# Autodesk Inventor assembly: S1702_EnsembleManetteTotal
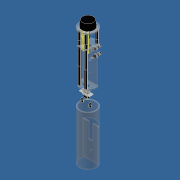
[picture p0: Inventor's stored thumbnail of the model, 180x180]
Saved by Autodesk Inventor 2015 SP2 (Build 190223200, 223)
## iProperties
Created: 2017-12-07
Part Number: S1702_EnsembleManetteTotal
Project: Nom Projet
Description: Ens. Nom Ensemble
Document SubType Name: Assembly
Designer: Benoit.CURCHOD2
Author: Benoit.CURCHOD2
## Documents named in this file (24)
- Z:\COMMUN\4. Projets\2. Projets PO\S1702_Circuit_sport\14_Conception 3D\Manette\Final\S1702_EnsembleManetteTotal.iam
- Z:\COMMUN\4. Projets\2. Projets PO\S1702_Circuit_sport\14_Conception 3D\Manette\Final\S1702_couverclebas.ipt
- Z:\COMMUN\4. Projets\2. Projets PO\S1702_Circuit_sport\14_Conception 3D\Manette\Final\Bouton poussoir NO.iam
- Z:\COMMUN\4. Projets\2. Projets PO\S1702_Circuit_sport\14_Conception 3D\Manette\Final\Bouton.ipt
- Z:\COMMUN\4. Projets\2. Projets PO\S1702_Circuit_sport\14_Conception 3D\Manette\Final\Capuchon.ipt
- Z:\COMMUN\4. Projets\2. Projets PO\S1702_Circuit_sport\14_Conception 3D\Manette\Final\Entretoise 12 x M3.ipt
- Z:\COMMUN\4. Projets\2. Projets PO\S1702_Circuit_sport\14_Conception 3D\Manette\Final\Entretoise 25.ipt
- Z:\COMMUN\4. Projets\2. Projets PO\S1702_Circuit_sport\14_Conception 3D\Manette\Final\Entretoise 50.ipt
- Z:\COMMUN\4. Projets\2. Projets PO\S1702_Circuit_sport\14_Conception 3D\Manette\Final\Molette.ipt
- Z:\COMMUN\4. Projets\2. Projets PO\S1702_Circuit_sport\14_Conception 3D\Manette\Final\Plaque électro.ipt
- Z:\COMMUN\4. Projets\2. Projets PO\S1702_Circuit_sport\14_Conception 3D\Manette\Final\Potentiomètre.ipt
- Z:\COMMUN\4. Projets\2. Projets PO\S1702_Circuit_sport\14_Conception 3D\Manette\Final\S1702_butee.ipt
- Z:\COMMUN\4. Projets\2. Projets PO\S1702_Circuit_sport\14_Conception 3D\Manette\Final\S1702_couverclehaut.ipt
- Z:\COMMUN\4. Projets\2. Projets PO\S1702_Circuit_sport\14_Conception 3D\Manette\Final\S1702_couverclerailressort.ipt
- Z:\COMMUN\4. Projets\2. Projets PO\S1702_Circuit_sport\14_Conception 3D\Manette\Final\S1702_couverclereplat.ipt
- Z:\COMMUN\4. Projets\2. Projets PO\S1702_Circuit_sport\14_Conception 3D\Manette\Final\S1702_paroiinterne.ipt
- Z:\COMMUN\4. Projets\2. Projets PO\S1702_Circuit_sport\14_Conception 3D\Manette\Final\S1702_replat.ipt
- Z:\COMMUN\4. Projets\2. Projets PO\S1702_Circuit_sport\14_Conception 3D\Manette\Final\S1702_tubeexterne.ipt
- P:\Projet\S1702_Circuit_Portes_Ouvertes\InventorManette\Fiche.ipt
- C:\Users\Benoit.CURCHOD2\Documents\Inventor\Content Center Files\R2015\fr-FR\AS 1237 (2.1)\AS 1237 - 3.ipt
- C:\Users\Benoit.CURCHOD2\Documents\Inventor\Content Center Files\R2015\fr-FR\ISO 4762(1)\ISO 4762 - M3 x 8DIN EN ISO.ipt
- C:\Users\Benoit.CURCHOD2\Documents\Inventor\Content Center Files\R2015\fr-FR\ISO 10642(2)\ISO 10642  - M3  x  8.ipt
- Z:\COMMUN\4. Projets\2. Projets PO\S1702_Circuit_sport\14_Conception 3D\Manette\Final\Entretoise_M3x6.ipt
- C:\Users\Alexandre.PICOTTE\Documents\Inventor\Content Center Files\R2015\fr-FR\D-Sub Male Crimp\D-Sub Male Crimp 9CKT.ipt
## Components (39 placed, 23 different names)
1. S1702_couverclebas:1 — Logement:4, Logement:6, Logement:31, Logement:33, Logement:34, Logement:35, Logement:36
2. Bouton poussoir NO:1 [sub-assembly] — Logement:24
3. Bouton:1 — Logement:11, Logement:23
4. Capuchon:1 — Logement:11
5. Entretoise 12 x M3:1 — Logement:9, Logement:10
6. Entretoise 25:1 — Logement:10
7. Entretoise 50:1 — Logement:6, Logement:7
8. Molette:1 — Logement:12, Logement:30
9. Plaque électro:1 — Placage:2, Placage:3, Placage:4
10. Potentiomètre:1 — Placage:1, Logement:29
11. S1702_butee:1 — Logement:12, Placage:8
12. S1702_couverclehaut:1 — Logement:27, Logement:28, Logement:29, Placage:2, Logement:30, Placage:8
13. S1702_couverclerailressort:1 — Logement:21, Logement:22, Logement:28, Placage:1
14. S1702_couverclereplat:1 — Logement:8, Logement:9, Logement:18, Logement:19, Logement:20, Logement:26, Placage:3, Placage:4, Placage:5, Affleurement:1, Placage:6, Placage:7, Logement:37, Logement:38
15. S1702_paroiinterne:1 — Logement:23, Logement:24, Placage:5, Affleurement:1, Placage:6, Placage:7, Affleurement:2, Logement:46
16. S1702_replat:1 — Placage:9, Placage:10
17. S1702_tubeexterne:1 — Placage:9, Placage:10, Logement:31, Affleurement:2
18. Entretoise 50:2 — Logement:5, Logement:8
19. Entretoise 50:3 — Logement:4, Logement:5
20. Entretoise 50:4 — Logement:7, Logement:26
21. Entretoise 12 x M3:2 — Logement:18
22. Entretoise 25:2 — Logement:22
23. Entretoise 12 x M3:3 — Logement:19
24. Entretoise 25:3
25. Entretoise 12 x M3:4 — Logement:20
26. Entretoise 25:4 — Logement:21, Logement:27
27. Fiche:1 — Logement:33, Logement:34, Logement:44, Logement:45
28. AS 1237 (2.1) 3:1 — Logement:35, Logement:42
29. AS 1237 (2.1) 3:2 — Logement:36, Logement:41
30. AS 1237 (2.1) 3:3 — Logement:37, Logement:39
31. AS 1237 (2.1) 3:4 — Logement:38, Logement:40
32. DIN EN ISO 4762 M3 x 8:1 — Logement:42
33. DIN EN ISO 4762 M3 x 8:2 — Logement:41
34. DIN EN ISO 4762 M3 x 8:3 — Logement:40
35. DIN EN ISO 4762 M3 x 8:4 — Logement:39
36. Entretoise_M3x6:1 — Logement:44
37. Entretoise_M3x6:2 — Logement:45
38. DIN EN ISO 10642 M3  x  8:2 — Logement:46
39. Sertissage mâle D-Sub D-Sub Male Crimp 9CKT:1
## Relationships (50: Insert 38, Mate 10, Flush 2)
- Logement:4 [Insert]: S1702_couverclebas:1 ↔ Entretoise 50:3
- Logement:5 [Insert]: Entretoise 50:2 ↔ Entretoise 50:3
- Logement:6 [Insert]: S1702_couverclebas:1 ↔ Entretoise 50:1
- Logement:7 [Insert]: Entretoise 50:1 ↔ Entretoise 50:4
- Logement:8 [Insert]: S1702_couverclereplat:1 ↔ Entretoise 50:2
- Logement:9 [Insert]: Entretoise 12 x M3:1 ↔ S1702_couverclereplat:1
- Logement:10 [Insert]: Entretoise 12 x M3:1 ↔ Entretoise 25:1
- Logement:11 [Insert]: Bouton:1 ↔ Capuchon:1
- Logement:12 [Insert]: Molette:1 ↔ S1702_butee:1
- [Insert]: Entretoise 12 x M3:2 ↔ Entretoise 25:2
- [Insert]: Entretoise 12 x M3:3 ↔ Entretoise 25:3
- [Insert]: Entretoise 12 x M3:4 ↔ Entretoise 25:4
- Logement:18 [Insert]: S1702_couverclereplat:1 ↔ Entretoise 12 x M3:2
- Logement:19 [Insert]: S1702_couverclereplat:1 ↔ Entretoise 12 x M3:3
- Logement:20 [Insert]: S1702_couverclereplat:1 ↔ Entretoise 12 x M3:4
- Logement:21 [Insert]: S1702_couverclerailressort:1 ↔ Entretoise 25:4
- Logement:22 [Insert]: S1702_couverclerailressort:1 ↔ Entretoise 25:2
- Logement:23 [Insert] (-20 mm): Bouton:1 ↔ S1702_paroiinterne:1
- Logement:24 [Insert] (-20 mm): Bouton poussoir NO:1 ↔ S1702_paroiinterne:1
- Logement:26 [Insert]: S1702_couverclereplat:1 ↔ Entretoise 50:4
- Logement:27 [Insert]: S1702_couverclehaut:1 ↔ Entretoise 25:4
- Logement:28 [Insert]: S1702_couverclehaut:1 ↔ S1702_couverclerailressort:1
- Placage:1 [Mate]: Potentiomètre:1 ↔ S1702_couverclerailressort:1
- Logement:29 [Insert]: Potentiomètre:1 ↔ S1702_couverclehaut:1
- Placage:2 [Mate]: Plaque électro:1 ↔ S1702_couverclehaut:1
- Placage:3 [Mate]: Plaque électro:1 ↔ S1702_couverclereplat:1
- Placage:4 [Mate]: Plaque électro:1 ↔ S1702_couverclereplat:1
- Placage:5 [Mate]: S1702_couverclereplat:1 ↔ S1702_paroiinterne:1
- Affleurement:1 [Flush]: S1702_couverclereplat:1 ↔ S1702_paroiinterne:1
- Placage:6 [Mate]: S1702_couverclereplat:1 ↔ S1702_paroiinterne:1
- Placage:7 [Mate]: S1702_couverclereplat:1 ↔ S1702_paroiinterne:1
- Logement:30 [Insert]: Molette:1 ↔ S1702_couverclehaut:1
- Placage:8 [Mate]: S1702_butee:1 ↔ S1702_couverclehaut:1
- Placage:9 [Mate]: S1702_replat:1 ↔ S1702_tubeexterne:1
- Placage:10 [Mate]: S1702_replat:1 ↔ S1702_tubeexterne:1
- Logement:31 [Insert] (-200 mm): S1702_couverclebas:1 ↔ S1702_tubeexterne:1
- Affleurement:2 [Flush]: S1702_paroiinterne:1 ↔ S1702_tubeexterne:1
- Logement:33 [Insert] (20 mm): S1702_couverclebas:1 ↔ Fiche:1
- Logement:34 [Insert] (20 mm): S1702_couverclebas:1 ↔ Fiche:1
- Logement:35 [Insert]: S1702_couverclebas:1 ↔ AS 1237 (2.1) 3:1
- Logement:36 [Insert]: S1702_couverclebas:1 ↔ AS 1237 (2.1) 3:2
- Logement:37 [Insert]: S1702_couverclereplat:1 ↔ AS 1237 (2.1) 3:3
- Logement:38 [Insert]: S1702_couverclereplat:1 ↔ AS 1237 (2.1) 3:4
- Logement:39 [Insert]: AS 1237 (2.1) 3:3 ↔ DIN EN ISO 4762 M3 x 8:4
- Logement:40 [Insert]: AS 1237 (2.1) 3:4 ↔ DIN EN ISO 4762 M3 x 8:3
- Logement:41 [Insert]: AS 1237 (2.1) 3:2 ↔ DIN EN ISO 4762 M3 x 8:2
- Logement:42 [Insert]: AS 1237 (2.1) 3:1 ↔ DIN EN ISO 4762 M3 x 8:1
- Logement:44 [Insert] (20 mm): Fiche:1 ↔ Entretoise_M3x6:1
- Logement:45 [Insert] (20 mm): Fiche:1 ↔ Entretoise_M3x6:2
- Logement:46 [Insert] (20 mm): S1702_paroiinterne:1 ↔ DIN EN ISO 10642 M3  x  8:2
## Named parameters: d14_d9 = 0 mm, d15_d9 = 0 mm, d16_d9 = 0 mm
